# Autodesk Inventor assembly: LauncherFullV1
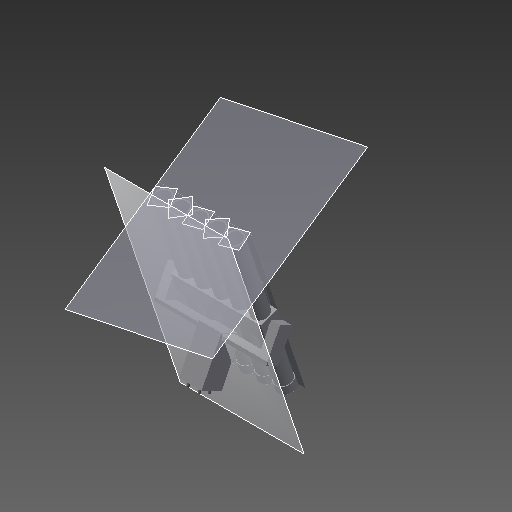
[picture p0: Inventor's stored thumbnail of the model, 512x512]
Saved by Autodesk Inventor 2019 (Build 230136000, 136)
## iProperties
Created: 2021-09-16
Part Number: LauncherFullV1
Document SubType Name: Assembly
Designer: timmy
Author: timmy
## Documents named in this file (4)
- S:\Inventor\RoboCatz\T-Shirt\LauncherFullV1.iam
- S:\Inventor\RoboCatz\T-Shirt\TubeHolderV2.ipt
- S:\Inventor\RoboCatz\T-Shirt\CannonV1.iam
- S:\Inventor\RoboCatz\T-Shirt\TubePostV1.ipt
## Components (7 placed, 3 different names)
1. TubeHolderV2:1 — Mate:1, Mate:2, Mate:3, Mate:4, Mate:5, Mate:6, Flush:12, Mate:7, Flush:13
2. CannonV1:1 [sub-assembly] — Mate:1, Flush:5, Flush:7, Flush:8, Flush:9, Flush:10, Flush:11, Flush:12
3. CannonV1:2 [sub-assembly] — Mate:2, Flush:1, Flush:2, Flush:7, Flush:8
4. CannonV1:3 [sub-assembly] — Mate:3, Flush:4, Flush:9
5. CannonV1:4 [sub-assembly] — Mate:4, Flush:6, Flush:10
6. CannonV1:5 [sub-assembly] — Mate:5, Flush:3, Flush:11
7. TubePostV1:1 — Mate:6, Mate:7, Angle:1
## Relationships (21: Flush 13, Mate 7, Angle 1)
- Mate:1: TubeHolderV2:1 ↔ CannonV1:1
- Mate:2: TubeHolderV2:1 ↔ CannonV1:2
- Mate:3: TubeHolderV2:1 ↔ CannonV1:3
- Mate:4: TubeHolderV2:1 ↔ CannonV1:4
- Mate:5: TubeHolderV2:1 ↔ CannonV1:5
- Flush:1: CannonV1:2
- Flush:2: CannonV1:2
- Flush:3: CannonV1:5
- Flush:4: CannonV1:3
- Flush:5: CannonV1:1
- Flush:6: CannonV1:4
- Mate:6: TubeHolderV2:1 ↔ TubePostV1:1
- Flush:7: CannonV1:1 ↔ CannonV1:2
- Flush:8: CannonV1:1 ↔ CannonV1:2
- Flush:9: CannonV1:1 ↔ CannonV1:3
- Flush:10: CannonV1:1 ↔ CannonV1:4
- Flush:11: CannonV1:1 ↔ CannonV1:5
- Flush:12: TubeHolderV2:1 ↔ CannonV1:1
- Mate:7: TubeHolderV2:1 ↔ TubePostV1:1
- Flush:13 (68.5546 mm): TubeHolderV2:1
- Angle:1 (225 deg): TubePostV1:1
